# Autodesk Inventor assembly: guidage_lineaire_shs25_lv_1_ss___2100l_30
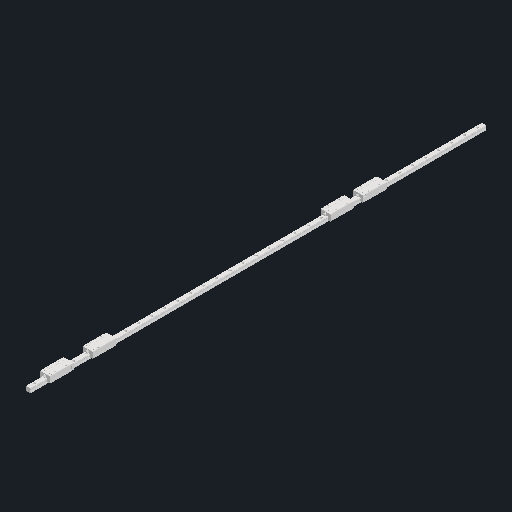
[picture p0: Inventor's stored thumbnail of the model, 512x512]
Saved by Autodesk Inventor 2025 (Build 290162000, 162)
## iProperties
Company: TraceParts S.A.
Created: 2024-05-17
Part Number: guidage_lineaire_shs25_lv_1_ss___2100l_30
Checked By: TraceParts S.A.
Catalog Web Link: www.traceparts.com
Document SubType Name: Assembly
Designer: TraceParts
Sending System: TraceParts v2
Major Version: 6.0
Minor Version: 0.0
Format Version: 0.0
Product Id: TraceParts v2
REFERENCE: SHS25 LV 1 SS + 2100L
SUPPLIER: THK
DESIGN: Linear guide SHS25LV type, 1 block(s), Without QZ lubricator, SS - With end, side, inner seals, Preload type: normal clearance, Rail length: 2100 mm, Accuracy grade: Normal grade, Symmetric G dimension: G=30mm
MASS: 7.39
TraceParts.PartNumber: 10-08102015-095416
TraceParts.PartVersion: 1.1.3
TraceParts.InstanceId: 10-08102015-0954166CH82IM0FDLAXH815O5G7ECGF
TraceParts.PartTitle: Caged Ball LM Guide Global Standard Size Model SHS-LV
TRACEPARTS: TRACEPARTS
TraceParts.PartLanguage: en
Author: TraceParts
## Documents named in this file (3)
- D:\UNAL\2024-1S\APM\Digital Factory\Linear Guides & Ball Screws\guidage_lineaire_shs25_lv_1_ss___2100l_30.iam
- D:\UNAL\2024-1S\APM\Digital Factory\Linear Guides & Ball Screws\guidage_lineaire_shs25_lv_1_ss___2100l_30_01.ipt
- D:\UNAL\2024-1S\APM\Digital Factory\Linear Guides & Ball Screws\guidage_lineaire_shs25_lv_1_ss___2100l_30_02.ipt
## Components (5 placed, 3 different names)
1. guidage_lineaire_shs25_lv_1_ss___2100l_30_Temp_1:1 — Slider:1, Slider:2, Slider:3, Slider:4
2. guidage_lineaire_shs25_lv_1_ss___2100l_30_Temp_2:1 — Slider:1
3. guidage_lineaire_shs25_lv_1_ss___2100l_30_02:2 — Slider:2
4. guidage_lineaire_shs25_lv_1_ss___2100l_30_02:3 — Slider:4
5. guidage_lineaire_shs25_lv_1_ss___2100l_30_02:4 — Slider:3
## Relationships (4: TranslationJoint 4)
- Slider:1 [TranslationJoint]: guidage_lineaire_shs25_lv_1_ss___2100l_30_Temp_1:1 ↔ guidage_lineaire_shs25_lv_1_ss___2100l_30_Temp_2:1
- Slider:2 [TranslationJoint]: guidage_lineaire_shs25_lv_1_ss___2100l_30_Temp_1:1 ↔ guidage_lineaire_shs25_lv_1_ss___2100l_30_02:2
- Slider:3 [TranslationJoint]: guidage_lineaire_shs25_lv_1_ss___2100l_30_Temp_1:1 ↔ guidage_lineaire_shs25_lv_1_ss___2100l_30_02:4
- Slider:4 [TranslationJoint]: guidage_lineaire_shs25_lv_1_ss___2100l_30_Temp_1:1 ↔ guidage_lineaire_shs25_lv_1_ss___2100l_30_02:3
